# Autodesk Inventor assembly: PneumaticWheel_am-0970
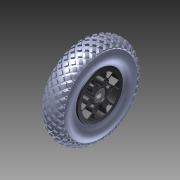
[picture p0: Inventor's stored thumbnail of the model, 180x180]
Saved by Autodesk Inventor 2013 SP1 (Build 170176100, 176)
## iProperties
Created: 2013-01-06
Part Number: PneumaticWheel_am-0970
Document SubType Name: Assembly
Designer: Moses
Mass: 459.953 g
Surface Area: 2436.37 cm^2
Volume: 459.953 cm^3
Density: 1 g/cm^3
Author: Moses
## Documents named in this file (5)
- C:\Users\Moses\Documents\Inventor\2013 Team 3061 Robot\Drivetrain\PneumaticWheel_am-0970\PneumaticWheel_am-0970.iam
- C:\Users\Moses\Documents\Inventor\2013 Team 3061 Robot\Drivetrain\PneumaticWheel_am-0970\Tire.ipt
- C:\Users\Moses\Documents\Inventor\2013 Team 3061 Robot\Drivetrain\PneumaticWheel_am-0970\Valve.ipt
- C:\Users\Moses\Documents\Inventor\2013 Team 3061 Robot\Drivetrain\PneumaticWheel_am-0970\Pneumatic Hub.iam
- C:\Users\Moses\Documents\Inventor\2013 Team 3061 Robot\Drivetrain\PneumaticWheel_am-0970\r8 bearing.ipt
## Components (5 placed, 4 different names)
1. Tire:1
2. Valve:1
3. Pneumatic Hub:1 [sub-assembly] — Insert:1, Insert:2
4. r8 bearing:1 — Insert:1
5. r8 bearing:2 — Insert:2
## Relationships (2: Insert 2)
- Insert:1: Pneumatic Hub:1 ↔ r8 bearing:1
- Insert:2: Pneumatic Hub:1 ↔ r8 bearing:2
